# Autodesk Inventor assembly: ENSAMBLE_CON_BRAZO
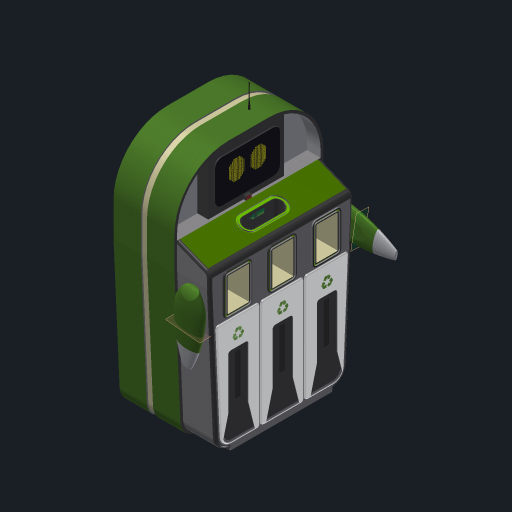
[picture p0: Inventor's stored thumbnail of the model, 512x512]
Saved by Autodesk Inventor 2024.3 (Build 283343000, 343)
## iProperties
Created: 2024-06-16
Part Number: ENSAMBLE_CON_BRAZO
Material: Generic
Document SubType Name: Assembly
Designer: Niler
Author: Niler
## Documents named in this file (4)
- C:\Users\Niler\OneDrive\Escritorio\RECICLADOR\RECICLADOR_MODELO_3D\VERSION_3\ENSAMBLE_CON_BRAZO.iam
- C:\Users\Niler\OneDrive\Escritorio\RECICLADOR\RECICLADOR_MODELO_3D\VERSION_3\CARCASA_V4 - Copy.ipt
- C:\Users\Niler\OneDrive\Escritorio\RECICLADOR\RECICLADOR_MODELO_3D\BRAZO.ipt
- C:\Users\Niler\OneDrive\Escritorio\RECICLADOR\RECICLADOR_MODELO_3D\ANTENA 433MHZ_VEHICULO.ipt
## Components (4 placed, 3 different names)
1. CARCASA_V4 - Copy:1 — Mate:1, Mate:2, Mate:3
2. BRAZO:1 — Mate:1
3. BRAZO:2 — Mate:2
4. ANTENA 433MHZ_VEHICULO:1 — Mate:3
## Relationships (3: Mate 3)
- Mate:1: CARCASA_V4 - Copy:1 ↔ BRAZO:1
- Mate:2: CARCASA_V4 - Copy:1 ↔ BRAZO:2
- Mate:3: CARCASA_V4 - Copy:1 ↔ ANTENA 433MHZ_VEHICULO:1
